# Autodesk Inventor assembly: StressAnalysisAssembly
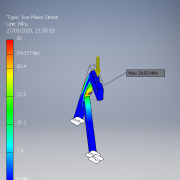
[picture p0: Inventor's stored thumbnail of the model, 180x180]
Saved by Autodesk Inventor 2018.3 (Build 223284000, 284)
## iProperties
Created: 2020-03-28
Part Number: StressAnalysisAssembly
Document SubType Name: Assembly
Designer: Ivan
Author: Ivan
## Documents named in this file (9)
- C:\Users\Ivan\Documents\GitHub\Tensegrity-Imposible-Table\3D model\StressAnalysisAssembly.iam
- C:\Users\Ivan\Documents\GitHub\Tensegrity-Imposible-Table\3D model\TableBaseWithHoles.ipt
- C:\Users\Ivan\Documents\GitHub\Tensegrity-Imposible-Table\3D model\TableSupport.ipt
- C:\Users\Ivan\Documents\GitHub\Tensegrity-Imposible-Table\3D model\StressAnalysisAssembly\AIP\FEA\d6zroh8xs.fins
- C:\Users\Ivan\Documents\GitHub\Tensegrity-Imposible-Table\3D model\StressAnalysisAssembly\AIP\FEA\d6zroh8xs.fsat
- C:\Users\Ivan\Documents\GitHub\Tensegrity-Imposible-Table\3D model\StressAnalysisAssembly\AIP\FEA\d6zroh8xs.ftes
- C:\Users\Ivan\Documents\GitHub\Tensegrity-Imposible-Table\3D model\StressAnalysisAssembly\AIP\FEA\d6zroh8xs.fwiz
- C:\Users\Ivan\Documents\GitHub\Tensegrity-Imposible-Table\3D model\StressAnalysisAssembly\AIP\FEA\d6zxomkcg.fmsh
- C:\Users\Ivan\Documents\GitHub\Tensegrity-Imposible-Table\3D model\StressAnalysisAssembly\AIP\FEA\d6zxomkch.fres
## Components (2 placed, 2 different names)
1. TableBaseWithHoles:1 — Mate:1, Mate:3, Mate:4
2. TableSupport:1 — Mate:1, Mate:3, Mate:4
## Relationships (3: Mate 3)
- Mate:1: TableBaseWithHoles:1 ↔ TableSupport:1
- Mate:3 (0.25 mm): TableBaseWithHoles:1 ↔ TableSupport:1
- Mate:4: TableBaseWithHoles:1 ↔ TableSupport:1
## Named parameters: sa_0 = -2.6e-12, sa_1 = 1.4e-12, sa_2 = -4000
note: some values were not read from the file. Shown as the stored number, unit unknown: "sa_0", "sa_1", "sa_2".
